# Autodesk Inventor assembly: 라즈베리파이 보관소
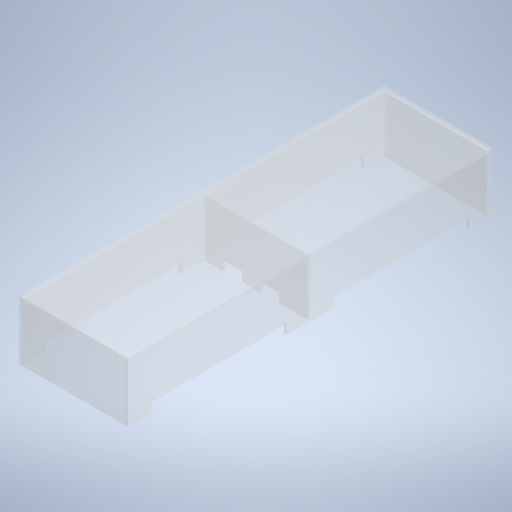
[picture p0: Inventor's stored thumbnail of the model, 512x512]
Saved by Autodesk Inventor 2024 (Build 280153000, 153)
## iProperties
Created: 2024-04-10
Part Number: 라즈베리파이 보관소
Document SubType Name: Assembly
Designer: kkamin5
Author: kkamin5
## Documents named in this file (5)
- C:\Users\kkamin5\OneDrive - UOS\문서\Inventor\EBS project\모델링최종\라즈베리파이 보관소.iam
- C:\Users\kkamin5\OneDrive - UOS\문서\Inventor\EBS project\모델링최종\라즈베리파이보관_옆판.ipt
- C:\Users\kkamin5\OneDrive - UOS\문서\Inventor\EBS project\모델링최종\라즈베리파이보관_윗판.ipt
- C:\Users\kkamin5\OneDrive - UOS\문서\Inventor\EBS project\모델링최종\발받침대받침옆판.ipt
- C:\Users\kkamin5\OneDrive - UOS\문서\Inventor\EBS project\모델링최종\발받침대받침옆판2.ipt
## Components (6 placed, 4 different names)
1. 라즈베리파이보관_옆판:1 — 메이트:4, 플러쉬:6, 플러쉬:7, 메이트:6, 메이트:8, 메이트:9
2. 라즈베리파이보관_윗판:1 — 메이트:1, 플러쉬:1, 메이트:2, 메이트:3, 플러쉬:5, 메이트:4, 플러쉬:6, 플러쉬:7, 메이트:5
3. 발받침대받침옆판:1 — 메이트:1, 플러쉬:1, 플러쉬:8, 메이트:6, 메이트:7
4. 발받침대받침옆판2:1 — 메이트:2, 메이트:9
5. 발받침대받침옆판:2 — 메이트:3, 플러쉬:5, 메이트:8
6. 라즈베리파이보관_옆판:2 — 플러쉬:8, 메이트:5, 메이트:7
## Relationships (14: Mate 9, Flush 5)
- 메이트:1 [Mate]: 라즈베리파이보관_윗판:1 ↔ 발받침대받침옆판:1
- 플러쉬:1 [Flush]: 라즈베리파이보관_윗판:1 ↔ 발받침대받침옆판:1
- 메이트:2 [Mate]: 라즈베리파이보관_윗판:1 ↔ 발받침대받침옆판2:1
- 메이트:3 [Mate]: 라즈베리파이보관_윗판:1 ↔ 발받침대받침옆판:2
- 플러쉬:5 [Flush]: 라즈베리파이보관_윗판:1 ↔ 발받침대받침옆판:2
- 메이트:4 [Mate]: 라즈베리파이보관_옆판:1 ↔ 라즈베리파이보관_윗판:1
- 플러쉬:6 [Flush]: 라즈베리파이보관_옆판:1 ↔ 라즈베리파이보관_윗판:1
- 플러쉬:7 [Flush]: 라즈베리파이보관_옆판:1 ↔ 라즈베리파이보관_윗판:1
- 플러쉬:8 [Flush]: 발받침대받침옆판:1 ↔ 라즈베리파이보관_옆판:2
- 메이트:5 [Mate]: 라즈베리파이보관_윗판:1 ↔ 라즈베리파이보관_옆판:2
- 메이트:6 [Mate]: 라즈베리파이보관_옆판:1 ↔ 발받침대받침옆판:1
- 메이트:7 [Mate]: 발받침대받침옆판:1 ↔ 라즈베리파이보관_옆판:2
- 메이트:8 [Mate]: 라즈베리파이보관_옆판:1 ↔ 발받침대받침옆판:2
- 메이트:9 [Mate]: 라즈베리파이보관_옆판:1 ↔ 발받침대받침옆판2:1
